# Autodesk Inventor assembly: Assembly2
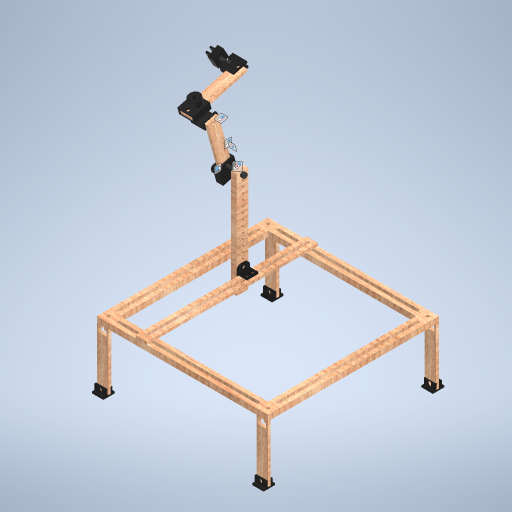
[picture p0: Inventor's stored thumbnail of the model, 512x512]
Saved by Autodesk Inventor 2023 (Build 270158000, 158)
## iProperties
Created: 2023-12-15
Part Number: Assembly2
Document SubType Name: Assembly
Designer: Mustapha
Author: Mustapha
## Documents named in this file (13)
- D:\EDU\Senior 2\Robotics\Activity\Assembly2.iam
- D:\EDU\Senior 2\Robotics\Activity\XYbase.ipt
- D:\EDU\Senior 2\Robotics\Activity\XYarm.ipt
- D:\EDU\Senior 2\Robotics\Activity\XY_Zfixer.ipt
- D:\EDU\Senior 2\Robotics\Activity\Zarm.ipt
- D:\EDU\Senior 2\Robotics\Activity\RollY.ipt
- D:\EDU\Senior 2\Robotics\Activity\RollYAxis.ipt
- D:\EDU\Senior 2\Robotics\Activity\M5 Hex Screw v2.ipt
- D:\EDU\Senior 2\Robotics\Activity\RollXAxisEnd.ipt
- D:\EDU\Senior 2\Robotics\Activity\RollYAxisEnd.ipt
- D:\EDU\Senior 2\Robotics\Activity\RollZ.ipt
- D:\EDU\Senior 2\Robotics\Activity\Leg1.ipt
- D:\EDU\Senior 2\Robotics\Activity\LegStablizer.ipt
## Components (22 placed, 12 different names)
1. XYbase:1 — Mate:1, Flush:1, Mate:21, Flush:6, Flush:7, Mate:22, Flush:8, Flush:9, Mate:23, Flush:10, Flush:11, Mate:24, Flush:12, Flush:13
2. XYarm:1 — Mate:1, Flush:1, Mate:2, Mate:3
3. XY_Zfixer:1 — Mate:2, Mate:3, Mate:4, Flush:2
4. Zarm:1 — Mate:4, Flush:2, Mate:7, Insert:1
5. RollY:1 — Mate:8, Angle:1, Mate:9
6. RollYAxis:1 — Mate:8, Angle:1, Mate:9, Rotational:1, Flush:4, Mate:15, Flush:5
7. M5 Hex Screw v2:1 — Mate:7, Insert:1, Rotational:1
8. RollXAxisEnd:1 — Flush:4, Mate:11, Mate:12, Mate:15, Flush:5
9. M5 Hex Screw v2:2 — Mate:11, Mate:12, Rotational:2
10. RollY:2 — Mate:13, Mate:14, Angle:2, Rotational:2
11. RollYAxis:2 — Mate:13, Mate:14, Angle:2, Mate:16, Mate:17, Angle:3
12. RollYAxisEnd:1 — Mate:16, Mate:17, Angle:3, Mate:18, Mate:19, Mate:20
13. RollZ:2 — Rotational:3
14. M5 Hex Screw v2:3 — Mate:18, Mate:19, Mate:20, Rotational:3
15. Leg1:1 — Mate:21, Flush:6, Flush:7, Mate:26, Flush:15
16. Leg1:2 — Mate:22, Flush:8, Flush:9, Mate:28, Flush:17
17. Leg1:3 — Mate:24, Flush:12, Flush:13, Mate:25, Flush:14
18. Leg1:4 — Mate:23, Flush:10, Flush:11, Mate:27, Flush:16
19. LegStablizer:1 — Mate:27, Flush:16
20. LegStablizer:2 — Mate:25, Flush:14
21. LegStablizer:3 — Mate:28, Flush:17
22. LegStablizer:4 — Mate:26, Flush:15
## Relationships (48: Mate 25, Flush 16, Angle 3, RevoluteJoint 3, Insert 1)
- Mate:1: XYbase:1 ↔ XYarm:1
- Flush:1: XYbase:1 ↔ XYarm:1
- Mate:2: XYarm:1 ↔ XY_Zfixer:1
- Mate:3: XYarm:1 ↔ XY_Zfixer:1
- Mate:4: XY_Zfixer:1 ↔ Zarm:1
- Flush:2: XY_Zfixer:1 ↔ Zarm:1
- Mate:7: Zarm:1 ↔ M5 Hex Screw v2:1
- Insert:1: Zarm:1 ↔ M5 Hex Screw v2:1
- Mate:8: RollY:1 ↔ RollYAxis:1
- Angle:1 (0 deg): RollY:1 ↔ RollYAxis:1
- Mate:9: RollY:1 ↔ RollYAxis:1
- Rotational:1 [RevoluteJoint]: RollYAxis:1 ↔ M5 Hex Screw v2:1
- Flush:4: RollYAxis:1 ↔ RollXAxisEnd:1
- Mate:11: RollXAxisEnd:1 ↔ M5 Hex Screw v2:2
- Mate:12: RollXAxisEnd:1 ↔ M5 Hex Screw v2:2
- Mate:13: RollY:2 ↔ RollYAxis:2
- Mate:14: RollY:2 ↔ RollYAxis:2
- Angle:2 (0 deg): RollY:2 ↔ RollYAxis:2
- Rotational:2 [RevoluteJoint]: M5 Hex Screw v2:2 ↔ RollY:2
- Mate:15: RollYAxis:1 ↔ RollXAxisEnd:1
- Flush:5 (-2 mm): RollYAxis:1 ↔ RollXAxisEnd:1
- Mate:16: RollYAxis:2 ↔ RollYAxisEnd:1
- Mate:17: RollYAxis:2 ↔ RollYAxisEnd:1
- Angle:3 (0 deg): RollYAxis:2 ↔ RollYAxisEnd:1
- Mate:18: RollYAxisEnd:1 ↔ M5 Hex Screw v2:3
- Mate:19 (-12.5 mm): RollYAxisEnd:1 ↔ M5 Hex Screw v2:3
- Mate:20 (-6 mm): RollYAxisEnd:1 ↔ M5 Hex Screw v2:3
- Rotational:3 [RevoluteJoint]: RollZ:2 ↔ M5 Hex Screw v2:3
- Mate:21: XYbase:1 ↔ Leg1:1
- Flush:6: XYbase:1 ↔ Leg1:1
- Flush:7: XYbase:1 ↔ Leg1:1
- Mate:22: XYbase:1 ↔ Leg1:2
- Flush:8: XYbase:1 ↔ Leg1:2
- Flush:9: XYbase:1 ↔ Leg1:2
- Mate:23: XYbase:1 ↔ Leg1:4
- Flush:10: XYbase:1 ↔ Leg1:4
- Flush:11: XYbase:1 ↔ Leg1:4
- Mate:24: XYbase:1 ↔ Leg1:3
- Flush:12: XYbase:1 ↔ Leg1:3
- Flush:13: XYbase:1 ↔ Leg1:3
- Mate:25: Leg1:3 ↔ LegStablizer:2
- Flush:14: Leg1:3 ↔ LegStablizer:2
- Mate:26: Leg1:1 ↔ LegStablizer:4
- Flush:15: Leg1:1 ↔ LegStablizer:4
- Mate:27: Leg1:4 ↔ LegStablizer:1
- Flush:16: Leg1:4 ↔ LegStablizer:1
- Mate:28: Leg1:2 ↔ LegStablizer:3
- Flush:17: Leg1:2 ↔ LegStablizer:3
